# Autodesk Inventor assembly: PlatformAssenm
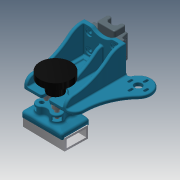
[picture p0: Inventor's stored thumbnail of the model, 180x180]
Saved by Autodesk Inventor 2014 (Build 180170000, 170)
## iProperties
Created: 2014-09-17
Part Number: PlatformAssenm
Document SubType Name: Assembly
Designer: Peele
Author: Peele
## Documents named in this file (7)
- E:\Copy\DLP\PandaPrint\SubAssem\PlatformAssenm.iam
- E:\Copy\DLP\PandaPrint\CustomParts\BuildMount.ipt
- E:\Copy\DLP\PandaPrint\CustomParts\PlateAttache.ipt
- E:\Copy\DLP\PandaPrint\StockParts\ThumbScrew.ipt
- E:\Copy\DLP\PandaPrint\StockParts\Knob.ipt
- E:\Copy\DLP\PandaPrint\StockParts\AluminumBlock.ipt
- E:\Copy\DLP\PandaPrint\StockParts\bLOCK.ipt
## Components (9 placed, 6 different names)
1. BuildMount:1 — Mate:1, Mate:2, Flush:1, Mate:9, Mate:10, Mate:13, Mate:22, Mate:23, Mate:24
2. PlateAttache:1 — Mate:14, Mate:15, Mate:16, Mate:17, Mate:19, Mate:21
3. ThumbScrew:1 — Flush:2, Flush:3, Flush:4, Mate:13, Mate:15, Mate:16
4. ThumbScrew:2 — Flush:3
5. ThumbScrew:3 — Flush:4, Mate:19
6. ThumbScrew:4 — Flush:2, Mate:17
7. Knob:1 — Mate:1, Mate:2, Mate:8, Mate:14
8. AluminumBlock:1 — Mate:8
9. bLOCK:1 — Mate:22, Mate:23, Mate:24
## Relationships (19: Mate 15, Flush 4)
- Mate:1: BuildMount:1 ↔ Knob:1
- Mate:2: BuildMount:1 ↔ Knob:1
- Mate:8: Knob:1 ↔ AluminumBlock:1
- Flush:1: BuildMount:1
- Mate:9: BuildMount:1
- Mate:10: BuildMount:1
- Flush:2: ThumbScrew:1 ↔ ThumbScrew:4
- Flush:3: ThumbScrew:1 ↔ ThumbScrew:2
- Flush:4: ThumbScrew:1 ↔ ThumbScrew:3
- Mate:13: BuildMount:1 ↔ ThumbScrew:1
- Mate:14: PlateAttache:1 ↔ Knob:1
- Mate:15 (5 mm): PlateAttache:1 ↔ ThumbScrew:1
- Mate:16: PlateAttache:1 ↔ ThumbScrew:1
- Mate:17: PlateAttache:1 ↔ ThumbScrew:4
- Mate:19: PlateAttache:1 ↔ ThumbScrew:3
- Mate:21: PlateAttache:1
- Mate:22: BuildMount:1 ↔ bLOCK:1
- Mate:23: BuildMount:1 ↔ bLOCK:1
- Mate:24: BuildMount:1 ↔ bLOCK:1
